# Autodesk Inventor assembly: Assembly3
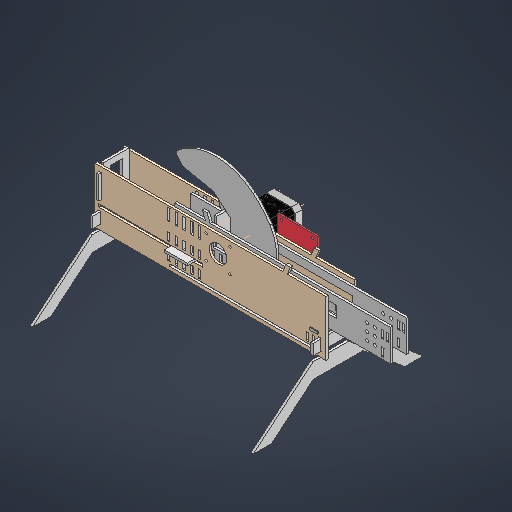
[picture p0: Inventor's stored thumbnail of the model, 512x512]
Saved by Autodesk Inventor 2027 (Build 310192000, 192)
## iProperties
Created: 2026-05-11
Part Number: Assembly3
Document SubType Name: Assembly
Designer: alexy
Author: alexy
## Documents named in this file (14)
- C:\Users\alexy\OneDrive\文件\group4\CarCourse_group4\SelfChosenTopic\Carinventor\2ndmodel\Assembly3-2.iam
- C:\Users\alexy\OneDrive\文件\group4\CarCourse_group4\SelfChosenTopic\Carinventor\2ndmodel\Sideboard3.ipt
- C:\Users\alexy\OneDrive\文件\group4\CarCourse_group4\SelfChosenTopic\Carinventor\2ndmodel\Nema 17 stepper motor.ipt
- C:\Users\alexy\OneDrive\文件\group4\CarCourse_group4\SelfChosenTopic\Carinventor\2ndmodel\Moving_rail3.ipt
- C:\Users\alexy\OneDrive\文件\group4\CarCourse_group4\SelfChosenTopic\Carinventor\2ndmodel\Middle_bar3.ipt
- C:\Users\alexy\OneDrive\文件\group4\CarCourse_group4\SelfChosenTopic\Carinventor\2ndmodel\contact_board3.ipt
- C:\Users\alexy\OneDrive\文件\group4\CarCourse_group4\SelfChosenTopic\Carinventor\2ndmodel\cam3-2.ipt
- C:\Users\alexy\OneDrive\文件\group4\CarCourse_group4\SelfChosenTopic\Carinventor\2ndmodel\Support_base.ipt
- C:\Users\alexy\OneDrive\文件\group4\CarCourse_group4\SelfChosenTopic\Carinventor\2ndmodel\Frontrail.ipt
- C:\Users\alexy\OneDrive\文件\group4\CarCourse_group4\SelfChosenTopic\Carinventor\2ndmodel\Back_board.ipt
- C:\Users\alexy\OneDrive\文件\group4\CarCourse_group4\SelfChosenTopic\Carinventor\2ndmodel\Battary_holder.ipt
- C:\Users\alexy\OneDrive\文件\group4\CarCourse_group4\SelfChosenTopic\Carinventor\2ndmodel\Battary_holder_part2.ipt
- C:\Users\alexy\OneDrive\文件\group4\CarCourse_group4\SelfChosenTopic\Carinventor\2ndmodel\Battary_holder_part3.ipt
- C:\Users\alexy\OneDrive\文件\group4\CarCourse_group4\SelfChosenTopic\Carinventor\2ndmodel\L298N.ipt
## Components (18 placed, 13 different names)
1. Sideboard3:1 — Mate:1, Insert:1, Angle:1, Mate:2, Mate:10, Mate:19, Mate:21, Mate:22, Mate:23, Mate:24, Mate:25, Mate:26, Flush:3, Flush:4, Mate:33, Mate:34, Mate:45, Mate:46, Mate:47, Mate:48, Mate:49, Mate:50
2. Nema 17 stepper motor:1 — Mate:1, Insert:1, Angle:1, Insert:2
3. Moving_rail3:1 — Mate:2, Mate:4, Mate:5, Mate:6, Mate:17
4. Middle_bar3:1 — Mate:4, Mate:5, Mate:6, Mate:10, Mate:11, Mate:12, Mate:13, Flush:1, Flush:2
5. contact_board3:2 — Mate:11, Mate:12, Mate:13
6. Middle_bar3:2 — Flush:1, Flush:2, Mate:17
7. cam3-2:1 — Insert:2
8. Sideboard3:3 — Flush:3, Flush:4, Mate:38
9. Support_base:1 — Mate:19, Mate:33, Mate:34
10. Frontrail:1 — Mate:21, Mate:22, Mate:23
11. Back_board:1 — Mate:24, Mate:25, Mate:26, Mate:38
12. Battary_holder:1 — Mate:42, Mate:43, Mate:44, Mate:45
13. Battary_holder:2 — Mate:35, Mate:36, Mate:37, Mate:39, Mate:40, Mate:41, Mate:47
14. Battary_holder_part2:1 — Mate:35, Mate:36, Mate:37, Mate:46
15. Battary_holder_part3:1 — Mate:39, Mate:40, Mate:41, Mate:42, Mate:43, Mate:44
16. contact_board3:3
17. L298N:1
18. Support_base:2 — Mate:48, Mate:49, Mate:50
## Relationships (42: Mate 35, Flush 4, Insert 2, Angle 1)
- Mate:1: Sideboard3:1 ↔ Nema 17 stepper motor:1
- Insert:1: Sideboard3:1 ↔ Nema 17 stepper motor:1
- Angle:1 (180 deg): Sideboard3:1 ↔ Nema 17 stepper motor:1
- Mate:2: Sideboard3:1 ↔ Moving_rail3:1
- Mate:4: Moving_rail3:1 ↔ Middle_bar3:1
- Mate:5: Moving_rail3:1 ↔ Middle_bar3:1
- Mate:6: Moving_rail3:1 ↔ Middle_bar3:1
- Mate:10 (3 mm): Sideboard3:1 ↔ Middle_bar3:1
- Mate:11: Middle_bar3:1 ↔ contact_board3:2
- Mate:12: Middle_bar3:1 ↔ contact_board3:2
- Mate:13: Middle_bar3:1 ↔ contact_board3:2
- Flush:1: Middle_bar3:1 ↔ Middle_bar3:2
- Flush:2: Middle_bar3:1 ↔ Middle_bar3:2
- Mate:17: Moving_rail3:1 ↔ Middle_bar3:2
- Insert:2 (10 mm): Nema 17 stepper motor:1 ↔ cam3-2:1
- Mate:19: Sideboard3:1 ↔ Support_base:1
- Mate:21: Sideboard3:1 ↔ Frontrail:1
- Mate:22: Sideboard3:1 ↔ Frontrail:1
- Mate:23: Sideboard3:1 ↔ Frontrail:1
- Mate:24: Sideboard3:1 ↔ Back_board:1
- Mate:25: Sideboard3:1 ↔ Back_board:1
- Mate:26: Sideboard3:1 ↔ Back_board:1
- Flush:3: Sideboard3:1 ↔ Sideboard3:3
- Flush:4: Sideboard3:1 ↔ Sideboard3:3
- Mate:33: Sideboard3:1 ↔ Support_base:1
- Mate:34: Sideboard3:1 ↔ Support_base:1
- Mate:35: Battary_holder:2 ↔ Battary_holder_part2:1
- Mate:36: Battary_holder:2 ↔ Battary_holder_part2:1
- Mate:37: Battary_holder:2 ↔ Battary_holder_part2:1
- Mate:38: Sideboard3:3 ↔ Back_board:1
- Mate:39: Battary_holder:2 ↔ Battary_holder_part3:1
- Mate:40: Battary_holder:2 ↔ Battary_holder_part3:1
- Mate:41: Battary_holder:2 ↔ Battary_holder_part3:1
- Mate:42: Battary_holder:1 ↔ Battary_holder_part3:1
- Mate:43: Battary_holder:1 ↔ Battary_holder_part3:1
- Mate:44: Battary_holder:1 ↔ Battary_holder_part3:1
- Mate:45: Sideboard3:1 ↔ Battary_holder:1
- Mate:46: Sideboard3:1 ↔ Battary_holder_part2:1
- Mate:47: Sideboard3:1 ↔ Battary_holder:2
- Mate:48: Sideboard3:1 ↔ Support_base:2
- Mate:49: Sideboard3:1 ↔ Support_base:2
- Mate:50: Sideboard3:1 ↔ Support_base:2
